# Autodesk Inventor assembly: Swerve-Drivetrain-2
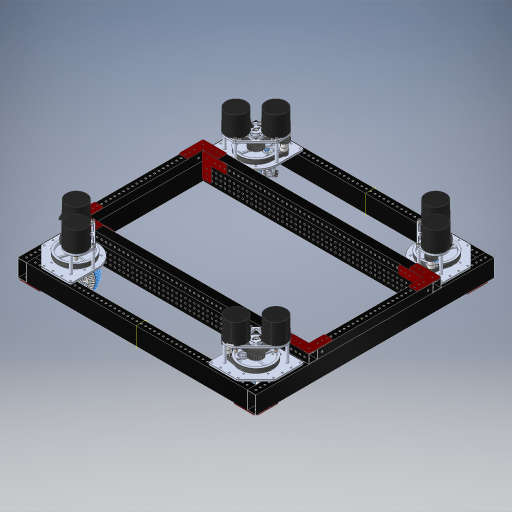
[picture p0: Inventor's stored thumbnail of the model, 512x512]
Saved by Autodesk Inventor 2024.2 (Build 282272000, 272)
## iProperties
Created: 2024-01-06
Part Number: Swerve-Drivetrain-2
Document SubType Name: Assembly
Designer: rohan
Author: rohan
## Documents named in this file (10)
- C:\Users\rohan\OneDrive - Hillsborough County Public Schools\Robotics\FIRST-Robotics-Competition\Crescendo\Minotaur-Crescendo-Robot\Swerve-Drivetrain-2.iam
- C:\Users\rohan\OneDrive - Hillsborough County Public Schools\Robotics\FIRST-Robotics-Competition\Crescendo\Minotaur-Crescendo-Robot\Motion\Swerve-Modules\MK3-Swerve-Module-Neos.iam
- C:\Users\rohan\OneDrive - Hillsborough County Public Schools\Robotics\FIRST-Robotics-Competition\Crescendo\Minotaur-Crescendo-Robot\Structure\MAXTube\2024-100-002-Front-Back-Extrusions.ipt
- C:\Users\rohan\OneDrive - Hillsborough County Public Schools\Robotics\FIRST-Robotics-Competition\Crescendo\Minotaur-Crescendo-Robot\Structure\MAXTube\2024-100-001-Left-Right-Extrusions.ipt
- C:\Users\rohan\OneDrive - Hillsborough County Public Schools\Robotics\FIRST-Robotics-Competition\Crescendo\Minotaur-Crescendo-Robot\Structure\MAXTube\2024-100-003-Middle-Extrusions.ipt
- C:\Users\rohan\OneDrive - Hillsborough County Public Schools\Robotics\FIRST-Robotics-Competition\Crescendo\Minotaur-Crescendo-Robot\Structure\Gussets\90-Degree-Sharp-Gusset.ipt
- C:\Users\rohan\OneDrive - Hillsborough County Public Schools\Robotics\FIRST-Robotics-Competition\Crescendo\Minotaur-Crescendo-Robot\Structure\Gussets\THRIFYBOT-L-Gusset.ipt
- C:\Users\rohan\OneDrive - Hillsborough County Public Schools\Robotics\FIRST-Robotics-Competition\Crescendo\Minotaur-Crescendo-Robot\Bumpers.ipt
- C:\Users\rohan\OneDrive - Hillsborough County Public Schools\Robotics\FIRST-Robotics-Competition\Crescendo\Minotaur-Crescendo-Robot\Structure\MAXTube\2024-100-004-Superstructure-Mount.ipt
- C:\Users\rohan\OneDrive - Hillsborough County Public Schools\Robotics\FIRST-Robotics-Competition\Crescendo\Minotaur-Crescendo-Robot\Structure\MAXTube\2024-100-004-Bumper-Mount.ipt
## Components (27 placed, 9 different names)
1. MK3-Swerve-Module-Neos:1 [sub-assembly] — Mate:10, Mate:56, Mate:57
2. MK3-Swerve-Module-Neos:2 [sub-assembly] — Mate:7, Mate:9, Mate:20
3. MK3-Swerve-Module-Neos:3 [sub-assembly] — Mate:4, Mate:16, Tangent:1, Mate:52, Mate:53
4. MK3-Swerve-Module-Neos:4 [sub-assembly] — Mate:1, Mate:2, Mate:3, Mate:14
5. 2024-100-002-Front-Back-Extrusions:1 — Mate:7, Mate:9, Mate:10, Mate:17, Flush:3, Flush:4, Mate:18, Flush:5, Mate:19, Flush:6, Symmetry:2, Mate:20, Mate:42, Mate:48, Mate:49, Mate:54, Mate:57, Mate:85
6. 2024-100-002-Front-Back-Extrusions:2 — Mate:1, Mate:2, Mate:3, Mate:4, Mate:13, Flush:1, Mate:15, Flush:2, Symmetry:2, Mate:40, Mate:41, Mate:44, Mate:45, Mate:46, Mate:47, Mate:52, Mate:53, Mate:66, Mate:88
7. 2024-100-001-Left-Right-Extrusions:1 — Mate:13, Mate:14, Flush:1, Symmetry:1, Mate:43
8. 2024-100-001-Left-Right-Extrusions:2 — Mate:15, Mate:16, Flush:2, Mate:17, Flush:3, Flush:4, Symmetry:1, Mate:55, Mate:56, Mate:67
9. 2024-100-003-Middle-Extrusions:1 — Mate:19, Flush:6, Symmetry:3, Mate:21, Flush:8, Mate:72, Mate:79, Mate:80, Mate:81, Mate:83
10. 2024-100-003-Middle-Extrusions:2 — Mate:18, Flush:5, Symmetry:3, Mate:21, Mate:69, Flush:7, Mate:76
11. 90-Degree-Sharp-Gusset:1 — Mate:42, Mate:54, Mate:55
12. 90-Degree-Sharp-Gusset:2 — Mate:43, Mate:48, Mate:49
13. 90-Degree-Sharp-Gusset:3 — Mate:41, Mate:44, Mate:45
14. 90-Degree-Sharp-Gusset:4 — Mate:40, Mate:46, Mate:47
15. Bumpers:1 — Mate:66, Mate:67, Mate:68, Mate:70, Mate:71, Mate:87, Mate:90
16. 2024-100-004-Superstructure-Mount:1 — Mate:69, Mate:70, Flush:7, Mate:73, Mate:74, Mate:75, Mate:77, Mate:78, Mate:97, Mate:98, Mate:100
17. 2024-100-004-Superstructure-Mount:2 — Flush:8, Mate:71, Mate:72, Mate:82, Mate:84, Mate:86, Mate:89, Mate:91, Mate:93, Insert:1
18. THRIFYBOT-L-Gusset:8 — Mate:80, Mate:81, Mate:82
19. THRIFYBOT-L-Gusset:9 — Mate:79, Mate:83, Mate:84
20. THRIFYBOT-L-Gusset:10 — Mate:74, Mate:77, Mate:78
21. THRIFYBOT-L-Gusset:11 — Mate:73, Mate:75, Mate:76
22. 2024-100-004-Bumper-Mount:1 — Mate:85, Mate:86, Mate:87, Mate:92, Mate:99
23. 2024-100-004-Bumper-Mount:2 — Mate:88, Mate:89, Mate:90, Mate:94, Mate:95, Mate:96, Mate:101
24. THRIFYBOT-L-Gusset:12 — Mate:91, Mate:92, Mate:93
25. THRIFYBOT-L-Gusset:13 — Mate:94, Insert:1, Mate:95
26. THRIFYBOT-L-Gusset:14 — Mate:97, Mate:98, Mate:99
27. THRIFYBOT-L-Gusset:15 — Mate:96, Mate:100, Mate:101
## Relationships (81: Mate 68, Flush 8, Symmetry 3, Tangent 1, Insert 1)
- Mate:1: MK3-Swerve-Module-Neos:4 ↔ 2024-100-002-Front-Back-Extrusions:2
- Mate:2: MK3-Swerve-Module-Neos:4 ↔ 2024-100-002-Front-Back-Extrusions:2
- Mate:3: MK3-Swerve-Module-Neos:4 ↔ 2024-100-002-Front-Back-Extrusions:2
- Mate:4: MK3-Swerve-Module-Neos:3 ↔ 2024-100-002-Front-Back-Extrusions:2
- Mate:7: MK3-Swerve-Module-Neos:2 ↔ 2024-100-002-Front-Back-Extrusions:1
- Mate:9: MK3-Swerve-Module-Neos:2 ↔ 2024-100-002-Front-Back-Extrusions:1
- Mate:10: MK3-Swerve-Module-Neos:1 ↔ 2024-100-002-Front-Back-Extrusions:1
- Mate:13: 2024-100-002-Front-Back-Extrusions:2 ↔ 2024-100-001-Left-Right-Extrusions:1
- Mate:14: MK3-Swerve-Module-Neos:4 ↔ 2024-100-001-Left-Right-Extrusions:1
- Flush:1: 2024-100-002-Front-Back-Extrusions:2 ↔ 2024-100-001-Left-Right-Extrusions:1
- Mate:15: 2024-100-002-Front-Back-Extrusions:2 ↔ 2024-100-001-Left-Right-Extrusions:2
- Mate:16: MK3-Swerve-Module-Neos:3 ↔ 2024-100-001-Left-Right-Extrusions:2
- Flush:2: 2024-100-002-Front-Back-Extrusions:2 ↔ 2024-100-001-Left-Right-Extrusions:2
- Mate:17: 2024-100-002-Front-Back-Extrusions:1 ↔ 2024-100-001-Left-Right-Extrusions:2
- Flush:3: 2024-100-002-Front-Back-Extrusions:1 ↔ 2024-100-001-Left-Right-Extrusions:2
- Flush:4: 2024-100-002-Front-Back-Extrusions:1 ↔ 2024-100-001-Left-Right-Extrusions:2
- Mate:18: 2024-100-002-Front-Back-Extrusions:1 ↔ 2024-100-003-Middle-Extrusions:2
- Flush:5: 2024-100-002-Front-Back-Extrusions:1 ↔ 2024-100-003-Middle-Extrusions:2
- Mate:19: 2024-100-002-Front-Back-Extrusions:1 ↔ 2024-100-003-Middle-Extrusions:1
- Flush:6: 2024-100-002-Front-Back-Extrusions:1 ↔ 2024-100-003-Middle-Extrusions:1
- Symmetry:1: 2024-100-001-Left-Right-Extrusions:1 ↔ 2024-100-001-Left-Right-Extrusions:2
- Symmetry:2: 2024-100-002-Front-Back-Extrusions:1 ↔ 2024-100-002-Front-Back-Extrusions:2
- Tangent:1: MK3-Swerve-Module-Neos:3
- Symmetry:3: 2024-100-003-Middle-Extrusions:1 ↔ 2024-100-003-Middle-Extrusions:2
- Mate:20: MK3-Swerve-Module-Neos:2 ↔ 2024-100-002-Front-Back-Extrusions:1
- Mate:21 (330.2 mm): 2024-100-003-Middle-Extrusions:1 ↔ 2024-100-003-Middle-Extrusions:2
- Mate:40: 2024-100-002-Front-Back-Extrusions:2 ↔ 90-Degree-Sharp-Gusset:4
- Mate:41: 2024-100-002-Front-Back-Extrusions:2 ↔ 90-Degree-Sharp-Gusset:3
- Mate:42: 2024-100-002-Front-Back-Extrusions:1 ↔ 90-Degree-Sharp-Gusset:1
- Mate:43: 2024-100-001-Left-Right-Extrusions:1 ↔ 90-Degree-Sharp-Gusset:2
- Mate:44: 2024-100-002-Front-Back-Extrusions:2 ↔ 90-Degree-Sharp-Gusset:3
- Mate:45: 2024-100-002-Front-Back-Extrusions:2 ↔ 90-Degree-Sharp-Gusset:3
- Mate:46: 2024-100-002-Front-Back-Extrusions:2 ↔ 90-Degree-Sharp-Gusset:4
- Mate:47: 2024-100-002-Front-Back-Extrusions:2 ↔ 90-Degree-Sharp-Gusset:4
- Mate:48: 2024-100-002-Front-Back-Extrusions:1 ↔ 90-Degree-Sharp-Gusset:2
- Mate:49: 2024-100-002-Front-Back-Extrusions:1 ↔ 90-Degree-Sharp-Gusset:2
- Mate:52: MK3-Swerve-Module-Neos:3 ↔ 2024-100-002-Front-Back-Extrusions:2
- Mate:53: MK3-Swerve-Module-Neos:3 ↔ 2024-100-002-Front-Back-Extrusions:2
- Mate:54: 2024-100-002-Front-Back-Extrusions:1 ↔ 90-Degree-Sharp-Gusset:1
- Mate:55: 2024-100-001-Left-Right-Extrusions:2 ↔ 90-Degree-Sharp-Gusset:1
- Mate:56: MK3-Swerve-Module-Neos:1 ↔ 2024-100-001-Left-Right-Extrusions:2
- Mate:57: MK3-Swerve-Module-Neos:1 ↔ 2024-100-002-Front-Back-Extrusions:1
- Mate:66: 2024-100-002-Front-Back-Extrusions:2 ↔ Bumpers:1
- Mate:67: 2024-100-001-Left-Right-Extrusions:2 ↔ Bumpers:1
- Mate:68 (38.1 mm): Bumpers:1
- Mate:69: 2024-100-003-Middle-Extrusions:2 ↔ 2024-100-004-Superstructure-Mount:1
- Mate:70: Bumpers:1 ↔ 2024-100-004-Superstructure-Mount:1
- Flush:7: 2024-100-003-Middle-Extrusions:2 ↔ 2024-100-004-Superstructure-Mount:1
- Flush:8: 2024-100-003-Middle-Extrusions:1 ↔ 2024-100-004-Superstructure-Mount:2
- Mate:71: Bumpers:1 ↔ 2024-100-004-Superstructure-Mount:2
- Mate:72: 2024-100-003-Middle-Extrusions:1 ↔ 2024-100-004-Superstructure-Mount:2
- Mate:73: 2024-100-004-Superstructure-Mount:1 ↔ THRIFYBOT-L-Gusset:11
- Mate:74: 2024-100-004-Superstructure-Mount:1 ↔ THRIFYBOT-L-Gusset:10
- Mate:75: 2024-100-004-Superstructure-Mount:1 ↔ THRIFYBOT-L-Gusset:11
- Mate:76: 2024-100-003-Middle-Extrusions:2 ↔ THRIFYBOT-L-Gusset:11
- Mate:77: 2024-100-004-Superstructure-Mount:1 ↔ THRIFYBOT-L-Gusset:10
- Mate:78: 2024-100-004-Superstructure-Mount:1 ↔ THRIFYBOT-L-Gusset:10
- Mate:79: 2024-100-003-Middle-Extrusions:1 ↔ THRIFYBOT-L-Gusset:9
- Mate:80: 2024-100-003-Middle-Extrusions:1 ↔ THRIFYBOT-L-Gusset:8
- Mate:81: 2024-100-003-Middle-Extrusions:1 ↔ THRIFYBOT-L-Gusset:8
- Mate:82: 2024-100-004-Superstructure-Mount:2 ↔ THRIFYBOT-L-Gusset:8
- Mate:83: 2024-100-003-Middle-Extrusions:1 ↔ THRIFYBOT-L-Gusset:9
- Mate:84: 2024-100-004-Superstructure-Mount:2 ↔ THRIFYBOT-L-Gusset:9
- Mate:85: 2024-100-002-Front-Back-Extrusions:1 ↔ 2024-100-004-Bumper-Mount:1
- Mate:86: 2024-100-004-Superstructure-Mount:2 ↔ 2024-100-004-Bumper-Mount:1
- Mate:87: Bumpers:1 ↔ 2024-100-004-Bumper-Mount:1
- Mate:88: 2024-100-002-Front-Back-Extrusions:2 ↔ 2024-100-004-Bumper-Mount:2
- Mate:89: 2024-100-004-Superstructure-Mount:2 ↔ 2024-100-004-Bumper-Mount:2
- Mate:90: Bumpers:1 ↔ 2024-100-004-Bumper-Mount:2
- Mate:91: 2024-100-004-Superstructure-Mount:2 ↔ THRIFYBOT-L-Gusset:12
- Mate:92: 2024-100-004-Bumper-Mount:1 ↔ THRIFYBOT-L-Gusset:12
- Mate:93: 2024-100-004-Superstructure-Mount:2 ↔ THRIFYBOT-L-Gusset:12
- Mate:94: 2024-100-004-Bumper-Mount:2 ↔ THRIFYBOT-L-Gusset:13
- Insert:1: 2024-100-004-Superstructure-Mount:2 ↔ THRIFYBOT-L-Gusset:13
- Mate:95: 2024-100-004-Bumper-Mount:2 ↔ THRIFYBOT-L-Gusset:13
- Mate:96: 2024-100-004-Bumper-Mount:2 ↔ THRIFYBOT-L-Gusset:15
- Mate:97: 2024-100-004-Superstructure-Mount:1 ↔ THRIFYBOT-L-Gusset:14
- Mate:98: 2024-100-004-Superstructure-Mount:1 ↔ THRIFYBOT-L-Gusset:14
- Mate:99: 2024-100-004-Bumper-Mount:1 ↔ THRIFYBOT-L-Gusset:14
- Mate:100: 2024-100-004-Superstructure-Mount:1 ↔ THRIFYBOT-L-Gusset:15
- Mate:101: 2024-100-004-Bumper-Mount:2 ↔ THRIFYBOT-L-Gusset:15
